# Autodesk Inventor assembly: Linear_guide
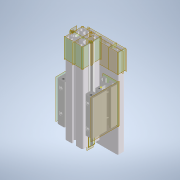
[picture p0: Inventor's stored thumbnail of the model, 180x180]
Saved by Autodesk Inventor 2022 (Build 260153000, 153)
## iProperties
Created: 2021-12-21
Part Number: Linear_guide
Document SubType Name: Assembly
Designer: matte
Author: matte
## Documents named in this file (9)
- C:\Users\matte\Documents\Mechanical Design Project\CAD\Linear_guide.iam
- C:\Users\matte\Documents\Mechanical Design Project\CAD\Inventor Component Part Files\01-Extrusion Profiles\01-40 series\10-040.ipt
- C:\Users\matte\Documents\Mechanical Design Project\CAD\Inventor Component Part Files\08-Linear Application\06-Linear Roller System\01-Roller System 6\30-404.ipt
- C:\Users\matte\Documents\Mechanical Design Project\CAD\Inventor Component Part Files\01-Extrusion Profiles\01-40 series\10-081.ipt
- C:\Users\matte\Documents\Mechanical Design Project\CAD\Inventor Component Part Files\08-Linear Application\06-Linear Roller System\01-Roller System 6\13-106.ipt
- C:\Users\matte\Documents\Mechanical Design Project\CAD\Inventor Component Part Files\08-Linear Application\06-Linear Roller System\01-Roller System 6\13-505.ipt
- C:\Users\matte\Documents\Mechanical Design Project\CAD\Inventor Component Part Files\08-Linear Application\06-Linear Roller System\01-Roller System 6\13-106_MIR.ipt
- C:\Users\matte\Documents\Mechanical Design Project\CAD\Inventor Component Part Files\08-Linear Application\06-Linear Roller System\01-Roller System 6\13-505_MIR.ipt
- C:\Users\matte\Documents\Mechanical Design Project\CAD\Inventor Component Part Files\08-Linear Application\06-Linear Roller System\01-Roller System 6\30-407.ipt
## Components (9 placed, 8 different names)
1. 10-040:1 — Coincidente:4, Coincidente:5, Allineato:5, Coincidente:6, Allineato:6, Allineato:7, Allineato:8, Coincidente:9, Coincidente:10, Coincidente:11, Allineato:10
2. 30-404:1 — Coincidente:1, Allineato:1, Allineato:11
3. 10-081:1 — Coincidente:1, Allineato:1, Coincidente:2, Allineato:3, Allineato:4, Coincidente:4, Coincidente:5
4. 30-404:2 — Coincidente:2, Allineato:3, Allineato:4, Allineato:11, Coincidente:12, Allineato:12, Allineato:13
5. 13-106:1 — Allineato:5, Coincidente:6, Allineato:6, Coincidente:7
6. 13-505:1 — Allineato:7, Allineato:8, Coincidente:7
7. 13-106_MIR:1 — Coincidente:8, Allineato:9, Coincidente:9, Coincidente:10, Allineato:10
8. 13-505_MIR:1 — Coincidente:8, Allineato:9, Coincidente:11
9. 30-407:1 — Coincidente:12, Allineato:12, Allineato:13
## Relationships (23: Flush 12, Mate 11)
- Coincidente:1 [Mate]: 30-404:1 ↔ 10-081:1
- Allineato:1 [Flush]: 30-404:1 ↔ 10-081:1
- Coincidente:2 [Mate]: 10-081:1 ↔ 30-404:2
- Allineato:3 [Flush]: 10-081:1 ↔ 30-404:2
- Allineato:4 [Flush] (60 mm): 10-081:1 ↔ 30-404:2
- Coincidente:4 [Mate] (40 mm): 10-040:1 ↔ 10-081:1
- Coincidente:5 [Mate] (-40 mm): 10-040:1 ↔ 10-081:1
- Allineato:5 [Flush]: 10-040:1 ↔ 13-106:1
- Coincidente:6 [Mate]: 10-040:1 ↔ 13-106:1
- Allineato:6 [Flush]: 10-040:1 ↔ 13-106:1
- Allineato:7 [Flush]: 10-040:1 ↔ 13-505:1
- Allineato:8 [Flush]: 10-040:1 ↔ 13-505:1
- Coincidente:7 [Mate]: 13-106:1 ↔ 13-505:1
- Coincidente:8 [Mate]: 13-106_MIR:1 ↔ 13-505_MIR:1
- Allineato:9 [Flush]: 13-106_MIR:1 ↔ 13-505_MIR:1
- Coincidente:9 [Mate]: 10-040:1 ↔ 13-106_MIR:1
- Coincidente:10 [Mate]: 10-040:1 ↔ 13-106_MIR:1
- Coincidente:11 [Mate]: 10-040:1 ↔ 13-505_MIR:1
- Allineato:10 [Flush]: 10-040:1 ↔ 13-106_MIR:1
- Allineato:11 [Flush]: 30-404:1 ↔ 30-404:2
- Coincidente:12 [Mate]: 30-404:2 ↔ 30-407:1
- Allineato:12 [Flush]: 30-404:2 ↔ 30-407:1
- Allineato:13 [Flush]: 30-404:2 ↔ 30-407:1
